# Autodesk Inventor assembly: ASSEMBLY_X_end
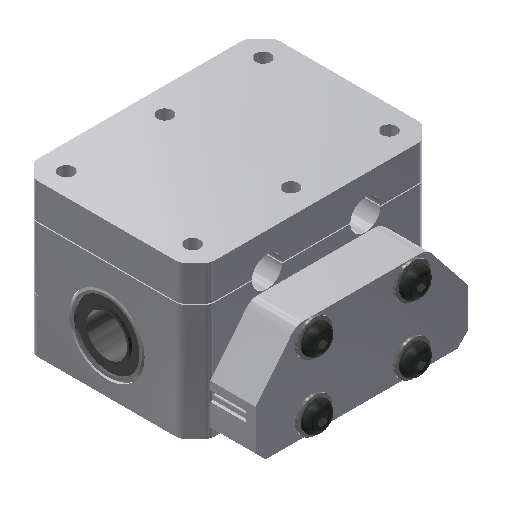
[picture p0: Inventor's stored thumbnail of the model, 512x512]
Saved by Autodesk Inventor 2026.1 (Build 301233000, 233)
## iProperties
Created: 2018-07-07
Part Number: ASSEMBLY_X_end
Document SubType Name: Assembly
Designer: Andrzej
Author: Andrzej
## Documents named in this file (8)
- C:\Users\Andrzej\OneDrive\_DRIVE_SYNCH_FILES\__ BYTECHLAB PROJECTS\MLTDIS - SMD Parts Sorting Machine\MCAD\1_REV1\ASSEMBLY_XY_AXIS_REVA\ASSEMBLY_X_end.iam
- C:\Users\Andrzej\OneDrive\_DRIVE_SYNCH_FILES\__ BYTECHLAB PROJECTS\MLTDIS - SMD Parts Sorting Machine\MCAD\1_REV1\ASSEMBLY_XY_AXIS_REVA\3DP_PLA_X_end_bottom_half.ipt
- C:\Users\Andrzej\OneDrive\_DRIVE_SYNCH_FILES\__ BYTECHLAB PROJECTS\MLTDIS - SMD Parts Sorting Machine\MCAD\1_REV1\ASSEMBLY_XY_AXIS_REVA\3DP_PLA_X_end_top_linear_shaft_clamp.ipt
- C:\Users\Andrzej\OneDrive\_DRIVE_SYNCH_FILES\__ BYTECHLAB PROJECTS\MLTDIS - SMD Parts Sorting Machine\MCAD\1_REV1\ASSEMBLY_XY_AXIS_REVA\3DP_PLA_X_end_top_half.ipt
- C:\Users\Andrzej\OneDrive\_DRIVE_SYNCH_FILES\__ BYTECHLAB PROJECTS\MLTDIS - SMD Parts Sorting Machine\MCAD\1_REV1\__COTS_PARTS\COTS_GENERIC_LM8UU_Linear_bearing.ipt
- C:\Users\Andrzej\OneDrive\_DRIVE_SYNCH_FILES\__ BYTECHLAB PROJECTS\MLTDIS - SMD Parts Sorting Machine\MCAD\1_REV1\ASSEMBLY_XY_AXIS_REVA\3DP_PLA_Y_axis_belt_mount.ipt
- C:\Users\Andrzej\OneDrive\_DRIVE_SYNCH_FILES\__ BYTECHLAB PROJECTS\MLTDIS - SMD Parts Sorting Machine\MCAD\1_REV1\__CONTENT_CENTER_PARTS\en-US\DIN 125-2  A\DIN 125-2 - A 3,2A.ipt
- C:\Users\Andrzej\OneDrive\_DRIVE_SYNCH_FILES\__ BYTECHLAB PROJECTS\MLTDIS - SMD Parts Sorting Machine\MCAD\1_REV1\__CONTENT_CENTER_PARTS\en-US\ISO 7380-1\ISO 7380-1 - M3 x 16.ipt
## Components (14 placed, 7 different names)
1. 3DP_PLA_X_end_bottom_half:1 — Mate:1, Flush:2, Flush:3, Mate:3, Mate:4, Flush:5, Mate:8, Flush:6, Mate:9
2. 3DP_PLA_X_end_top_linear_shaft_clamp:1 — Mate:2, Flush:1, Flush:4
3. 3DP_PLA_X_end_top_half:1 — Mate:1, Mate:2, Flush:1, Flush:2, Flush:3, Flush:4
4. COTS_GENERIC_LM8UU_Linear_bearing:1 — Mate:3, Mate:5
5. COTS_GENERIC_LM8UU_Linear_bearing:2 — Mate:4, Mate:5, Flush:5
6. 3DP_PLA_Y_axis_belt_mount:1 — Mate:8, Flush:6, Mate:9, Insert:1, Insert:2, Insert:3, Insert:4
7. DIN 125-2 A A 3,2:1 — Insert:1, Insert:5
8. DIN 125-2 A A 3,2:2 — Insert:2, Insert:6
9. DIN 125-2 A A 3,2:3 — Insert:3, Insert:7
10. DIN 125-2 A A 3,2:4 — Insert:4, Insert:8
11. ISO 7380-1 M3 x 16:1 — Insert:5
12. ISO 7380-1 M3 x 16:2 — Insert:6
13. ISO 7380-1 M3 x 16:3 — Insert:7
14. ISO 7380-1 M3 x 16:4 — Insert:8
## Relationships (21: Insert 8, Mate 7, Flush 6)
- Mate:1: 3DP_PLA_X_end_bottom_half:1 ↔ 3DP_PLA_X_end_top_half:1
- Mate:2 (0.2 mm): 3DP_PLA_X_end_top_linear_shaft_clamp:1 ↔ 3DP_PLA_X_end_top_half:1
- Flush:1: 3DP_PLA_X_end_top_linear_shaft_clamp:1 ↔ 3DP_PLA_X_end_top_half:1
- Flush:2: 3DP_PLA_X_end_bottom_half:1 ↔ 3DP_PLA_X_end_top_half:1
- Flush:3: 3DP_PLA_X_end_bottom_half:1 ↔ 3DP_PLA_X_end_top_half:1
- Flush:4: 3DP_PLA_X_end_top_linear_shaft_clamp:1 ↔ 3DP_PLA_X_end_top_half:1
- Mate:3: 3DP_PLA_X_end_bottom_half:1 ↔ COTS_GENERIC_LM8UU_Linear_bearing:1
- Mate:4: 3DP_PLA_X_end_bottom_half:1 ↔ COTS_GENERIC_LM8UU_Linear_bearing:2
- Mate:5: COTS_GENERIC_LM8UU_Linear_bearing:1 ↔ COTS_GENERIC_LM8UU_Linear_bearing:2
- Flush:5: 3DP_PLA_X_end_bottom_half:1 ↔ COTS_GENERIC_LM8UU_Linear_bearing:2
- Mate:8: 3DP_PLA_X_end_bottom_half:1 ↔ 3DP_PLA_Y_axis_belt_mount:1
- Flush:6: 3DP_PLA_X_end_bottom_half:1 ↔ 3DP_PLA_Y_axis_belt_mount:1
- Mate:9: 3DP_PLA_X_end_bottom_half:1 ↔ 3DP_PLA_Y_axis_belt_mount:1
- Insert:1: 3DP_PLA_Y_axis_belt_mount:1 ↔ DIN 125-2 A A 3,2:1
- Insert:2: 3DP_PLA_Y_axis_belt_mount:1 ↔ DIN 125-2 A A 3,2:2
- Insert:3: 3DP_PLA_Y_axis_belt_mount:1 ↔ DIN 125-2 A A 3,2:3
- Insert:4: 3DP_PLA_Y_axis_belt_mount:1 ↔ DIN 125-2 A A 3,2:4
- Insert:5: DIN 125-2 A A 3,2:1 ↔ ISO 7380-1 M3 x 16:1
- Insert:6: DIN 125-2 A A 3,2:2 ↔ ISO 7380-1 M3 x 16:2
- Insert:7: DIN 125-2 A A 3,2:3 ↔ ISO 7380-1 M3 x 16:3
- Insert:8: DIN 125-2 A A 3,2:4 ↔ ISO 7380-1 M3 x 16:4
